# Autodesk Inventor assembly: 8-mecanum-right-with-roller with hub
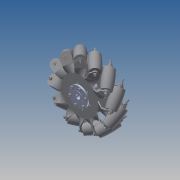
[picture p0: Inventor's stored thumbnail of the model, 180x180]
Saved by Autodesk Inventor 2014 SP1 (Build 180222100, 222)
## iProperties
Created: 2014-01-16
Part Number: 8-mecanum-right-with-roller with hub
Document SubType Name: Assembly
Designer: Pradhan Alexander
Author: Unknown
Title: //Amserv/amserver/AndyMark/Products/Wheel Mecanum/8 Mecanum Wheel/8 mecanum right with roller.stp
Organization: Unknown
Description: Unknown
Sending System: Unknown
Preprocessor: XStep 1.0
Author: Pradhan Alexander
## Documents named in this file (10)
- K:\MHS\Technology\Holliday B\Group Projects\Robotics\CAD Team\CAD Team 2014\Chassis 2014\8-mecanum-right-with-roller with hub.iam
- K:\MHS\Technology\Holliday B\Group Projects\Robotics\CAD Team\CAD Team 2014\Chassis 2014\Imported Components\8-mecanum-right-with-roller\washer0.ipt
- K:\MHS\Technology\Holliday B\Group Projects\Robotics\CAD Team\CAD Team 2014\Chassis 2014\Imported Components\8-mecanum-right-with-roller\#10 LockNut1.ipt
- K:\MHS\Technology\Holliday B\Group Projects\Robotics\CAD Team\CAD Team 2014\Chassis 2014\Imported Components\8-mecanum-right-with-roller\MBC Bushing MU04TH4.ipt
- K:\MHS\Technology\Holliday B\Group Projects\Robotics\CAD Team\CAD Team 2014\Chassis 2014\Imported Components\8-mecanum-right-with-roller\Mid Roller III2.ipt
- K:\MHS\Technology\Holliday B\Group Projects\Robotics\CAD Team\CAD Team 2014\Chassis 2014\Imported Components\8-mecanum-right-with-roller\SHCS 10-32x3_SHCS 10-32x4.ipt
- K:\MHS\Technology\Holliday B\Group Projects\Robotics\CAD Team\CAD Team 2014\Chassis 2014\Imported Components\8-mecanum-right-with-roller\Middle Axle3.ipt
- K:\MHS\Technology\Holliday B\Group Projects\Robotics\CAD Team\CAD Team 2014\Chassis 2014\Imported Components\8-mecanum-right-with-roller\Spacer AA.ipt
- K:\MHS\Technology\Holliday B\Group Projects\Robotics\CAD Team\CAD Team 2014\Chassis 2014\Imported Components\8-mecanum-right-with-roller\8 Mecanum Plate Right.ipt
- K:\MHS\Technology\Holliday B\Group Projects\Robotics\CAD Team\CAD Team 2014\Chassis 2014\Imported Components\am-0077a-500 Key Hub r2\am-0077a-500 Key Hub r2.ipt
## Components (118 placed, 9 different names)
1. washer0
2. washer0:1
3. washer0:2
4. washer0:3
5. washer0:4
6. washer0:5
7. washer0:6
8. washer0:7
9. washer0:8
10. washer0:9
11. washer0:10
12. washer0:11
13. washer0:12
14. washer0:13
15. washer0:14
16. washer0:15
17. washer0:16
18. washer0:17
19. washer0:18
20. washer0:19
21. washer0:20
22. washer0:21
23. washer0:22
24. washer0:23
25. #10 LockNut1
26. #10 LockNut1:1
27. #10 LockNut1:2
28. #10 LockNut1:3
29. #10 LockNut1:4
30. #10 LockNut1:5 — Insert:13
31. #10 LockNut1:6
32. #10 LockNut1:7
33. #10 LockNut1:8 — Insert:14
34. #10 LockNut1:9
35. #10 LockNut1:10
36. #10 LockNut1:11
37. #10 LockNut1:12 — Insert:12
38. #10 LockNut1:13 — Insert:11
39. #10 LockNut1:14 — Insert:15
40. #10 LockNut1:15
41. #10 LockNut1:16
42. #10 LockNut1:17 — Insert:16
43. MBC Bushing MU04TH4
44. MBC Bushing MU04TH4:1
45. MBC Bushing MU04TH4:2
46. MBC Bushing MU04TH4:3
47. MBC Bushing MU04TH4:4
48. MBC Bushing MU04TH4:5
49. MBC Bushing MU04TH4:6
50. MBC Bushing MU04TH4:7
51. MBC Bushing MU04TH4:8
52. MBC Bushing MU04TH4:9
53. MBC Bushing MU04TH4:10
54. MBC Bushing MU04TH4:11
55. MBC Bushing MU04TH4:12
56. MBC Bushing MU04TH4:13
57. MBC Bushing MU04TH4:14
58. MBC Bushing MU04TH4:15
59. MBC Bushing MU04TH4:16
60. MBC Bushing MU04TH4:17
61. MBC Bushing MU04TH4:18
62. MBC Bushing MU04TH4:19
63. MBC Bushing MU04TH4:20
64. MBC Bushing MU04TH4:21
65. MBC Bushing MU04TH4:22
66. MBC Bushing MU04TH4:23
67. Mid Roller III2
68. Mid Roller III2:1
69. Mid Roller III2:2
70. Mid Roller III2:3
71. Mid Roller III2:4
72. Mid Roller III2:5
73. Mid Roller III2:6
74. Mid Roller III2:7
75. Mid Roller III2:8
76. Mid Roller III2:9
77. Mid Roller III2:10
78. Mid Roller III2:11
79. SHCS 10-32x3_SHCS 10-32x4
80. SHCS 10-32x3_SHCS 10-32x4:1 — Insert:10
81. SHCS 10-32x3_SHCS 10-32x4:2 — Insert:8
82. SHCS 10-32x3_SHCS 10-32x4:3
83. SHCS 10-32x3_SHCS 10-32x4:4
84. SHCS 10-32x3_SHCS 10-32x4:5 — Insert:9
85. SHCS 10-32x3_SHCS 10-32x4:6 — Insert:5
86. SHCS 10-32x3_SHCS 10-32x4:7 — Insert:6
87. SHCS 10-32x3_SHCS 10-32x4:8
88. SHCS 10-32x3_SHCS 10-32x4:9
89. SHCS 10-32x3_SHCS 10-32x4:10
90. SHCS 10-32x3_SHCS 10-32x4:11
91. SHCS 10-32x3_SHCS 10-32x4:12
92. SHCS 10-32x3_SHCS 10-32x4:13
93. SHCS 10-32x3_SHCS 10-32x4:14
94. SHCS 10-32x3_SHCS 10-32x4:15 — Insert:7
95. SHCS 10-32x3_SHCS 10-32x4:16
96. SHCS 10-32x3_SHCS 10-32x4:17
97. Middle Axle3
98. Middle Axle3:1
99. Middle Axle3:2
100. Middle Axle3:3
101. Middle Axle3:4
102. Middle Axle3:5
103. Middle Axle3:6
104. Middle Axle3:7
105. Middle Axle3:8
106. Middle Axle3:9
107. Middle Axle3:10
108. Middle Axle3:11
109. Spacer AA
110. Spacer AA:1
111. Spacer AA:2
112. Spacer AA:3
113. Spacer AA:4
114. Spacer AA:5
115. 8 Mecanum Plate Right — Insert:1, Insert:2
116. 8 Mecanum Plate Right:1 — Insert:3, Insert:4
117. am-0077a-500 Key Hub r2:1 — Insert:1, Insert:2, Insert:5, Insert:6, Insert:7, Insert:8, Insert:9, Insert:10
118. am-0077a-500 Key Hub r2:2 — Insert:3, Insert:4, Insert:11, Insert:12, Insert:13, Insert:14, Insert:15, Insert:16
## Relationships (16: Insert 16)
- Insert:1: 8 Mecanum Plate Right ↔ am-0077a-500 Key Hub r2:1
- Insert:2: 8 Mecanum Plate Right ↔ am-0077a-500 Key Hub r2:1
- Insert:3: 8 Mecanum Plate Right:1 ↔ am-0077a-500 Key Hub r2:2
- Insert:4: 8 Mecanum Plate Right:1 ↔ am-0077a-500 Key Hub r2:2
- Insert:5: SHCS 10-32x3_SHCS 10-32x4:6 ↔ am-0077a-500 Key Hub r2:1
- Insert:6: SHCS 10-32x3_SHCS 10-32x4:7 ↔ am-0077a-500 Key Hub r2:1
- Insert:7: SHCS 10-32x3_SHCS 10-32x4:15 ↔ am-0077a-500 Key Hub r2:1
- Insert:8: SHCS 10-32x3_SHCS 10-32x4:2 ↔ am-0077a-500 Key Hub r2:1
- Insert:9: SHCS 10-32x3_SHCS 10-32x4:5 ↔ am-0077a-500 Key Hub r2:1
- Insert:10: SHCS 10-32x3_SHCS 10-32x4:1 ↔ am-0077a-500 Key Hub r2:1
- Insert:11: #10 LockNut1:13 ↔ am-0077a-500 Key Hub r2:2
- Insert:12: #10 LockNut1:12 ↔ am-0077a-500 Key Hub r2:2
- Insert:13: #10 LockNut1:5 ↔ am-0077a-500 Key Hub r2:2
- Insert:14: #10 LockNut1:8 ↔ am-0077a-500 Key Hub r2:2
- Insert:15: #10 LockNut1:14 ↔ am-0077a-500 Key Hub r2:2
- Insert:16: #10 LockNut1:17 ↔ am-0077a-500 Key Hub r2:2
